# Autodesk Inventor assembly: Assembly
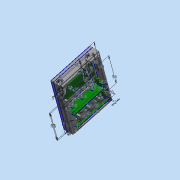
[picture p0: Inventor's stored thumbnail of the model, 180x180]
Saved by Autodesk Inventor 2015 (Build 190159000, 159)
## iProperties
Created: 2014-12-25
Part Number: Assembly
Document SubType Name: Assembly
Designer: Openlab
Author: Openlab
## Documents named in this file (6)
- C:\Users\Openlab\Documents\Alexey\HS-Spectrophotometer\parts\Assembly.iam
- C:\Users\Openlab\Documents\Alexey\HS-Spectrophotometer\parts\Base_V1.ipt
- C:\Users\Openlab\Documents\Alexey\HS-Spectrophotometer\parts\Motherboard_dummy.ipt
- C:\Users\Openlab\Documents\Alexey\HS-Spectrophotometer\parts\Sensor_Board_dummy.ipt
- C:\Users\Openlab\Documents\Alexey\HS-Spectrophotometer\parts\Led_Board_V1.ipt
- C:\Users\Openlab\Documents\Alexey\HS-Spectrophotometer\parts\filter.ipt
## Components (6 placed, 5 different names)
1. Base_V1:1 — Mate:1, Mate:4, Mate:8, Mate:12, Mate:14, Mate:16, Mate:17, Mate:18, Mate:19, Mate:21, Mate:22, Mate:23, Mate:24, Mate:25, Mate:26, Mate:27
2. Motherboard_dummy:1 — Mate:1, Mate:21, Mate:22, Mate:23
3. Sensor_Board_dummy:1 — Mate:4, Mate:8, Mate:25
4. Led_Board_V1:1 — Mate:18, Mate:19, Mate:24
5. filter:1 — Mate:12, Mate:17, Mate:26
6. filter:2 — Mate:14, Mate:16, Mate:27
## Relationships (16: Mate 16)
- Mate:1: Base_V1:1 ↔ Motherboard_dummy:1
- Mate:4: Base_V1:1 ↔ Sensor_Board_dummy:1
- Mate:8: Base_V1:1 ↔ Sensor_Board_dummy:1
- Mate:12: Base_V1:1 ↔ filter:1
- Mate:14: Base_V1:1 ↔ filter:2
- Mate:16: Base_V1:1 ↔ filter:2
- Mate:17: Base_V1:1 ↔ filter:1
- Mate:18: Base_V1:1 ↔ Led_Board_V1:1
- Mate:19: Base_V1:1 ↔ Led_Board_V1:1
- Mate:21: Base_V1:1 ↔ Motherboard_dummy:1
- Mate:22: Base_V1:1 ↔ Motherboard_dummy:1
- Mate:23: Base_V1:1 ↔ Motherboard_dummy:1
- Mate:24: Base_V1:1 ↔ Led_Board_V1:1
- Mate:25: Base_V1:1 ↔ Sensor_Board_dummy:1
- Mate:26: Base_V1:1 ↔ filter:1
- Mate:27: Base_V1:1 ↔ filter:2
